# Autodesk Inventor assembly: 階梯組合
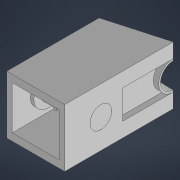
[picture p0: Inventor's stored thumbnail of the model, 180x180]
Saved by Autodesk Inventor 2021 (Build 250183000, 183)
## iProperties
Created: 2020-12-30
Part Number: 階梯組合
Document SubType Name: Assembly
Designer: zihon
Author: zihon
## Documents named in this file (7)
- C:\Users\zihon\Desktop\New folder\階梯組合.iam
- C:\Users\zihon\Desktop\New folder\架無軌道.ipt
- C:\Users\zihon\Desktop\New folder\零件1.ipt
- C:\Users\zihon\Desktop\New folder\零件2.ipt
- C:\Users\zihon\Desktop\New folder\零件3.ipt
- C:\Users\zihon\Desktop\New folder\零件4.ipt
- C:\Users\zihon\Desktop\New folder\軸.ipt
## Components (6 placed, 6 different names)
1. 架無軌道:1 — 齊平:1, 齊平:2, 齊平:3, 貼合:1, 貼合:2, 貼合:3, 貼合:4, 貼合:5, 貼合:6, 貼合:7, 貼合:8, 貼合:9, 齊平:4
2. 零件1:1 — 貼合:1, 貼合:5, 相切:1
3. 零件2:1 — 貼合:2, 貼合:6, 相切:2
4. 零件3:1 — 貼合:3, 貼合:7, 相切:3
5. 零件4:1 — 貼合:4, 貼合:8, 相切:4
6. 軸:1 — 貼合:9, 齊平:4, 相切:1, 相切:2, 相切:3, 相切:4
## Relationships (17: Mate 9, Flush 4, Tangent 4)
- 齊平:1 [Flush]: 架無軌道:1
- 齊平:2 [Flush]: 架無軌道:1
- 齊平:3 [Flush]: 架無軌道:1
- 貼合:1 [Mate]: 架無軌道:1 ↔ 零件1:1
- 貼合:2 [Mate]: 架無軌道:1 ↔ 零件2:1
- 貼合:3 [Mate]: 架無軌道:1 ↔ 零件3:1
- 貼合:4 [Mate]: 架無軌道:1 ↔ 零件4:1
- 貼合:5 [Mate]: 架無軌道:1 ↔ 零件1:1
- 貼合:6 [Mate]: 架無軌道:1 ↔ 零件2:1
- 貼合:7 [Mate]: 架無軌道:1 ↔ 零件3:1
- 貼合:8 [Mate]: 架無軌道:1 ↔ 零件4:1
- 貼合:9 [Mate]: 架無軌道:1 ↔ 軸:1
- 齊平:4 [Flush]: 架無軌道:1 ↔ 軸:1
- 相切:1 [Tangent]: 零件1:1 ↔ 軸:1
- 相切:2 [Tangent]: 零件2:1 ↔ 軸:1
- 相切:3 [Tangent]: 零件3:1 ↔ 軸:1
- 相切:4 [Tangent]: 零件4:1 ↔ 軸:1
